# Autodesk Inventor assembly: Assy_wrist
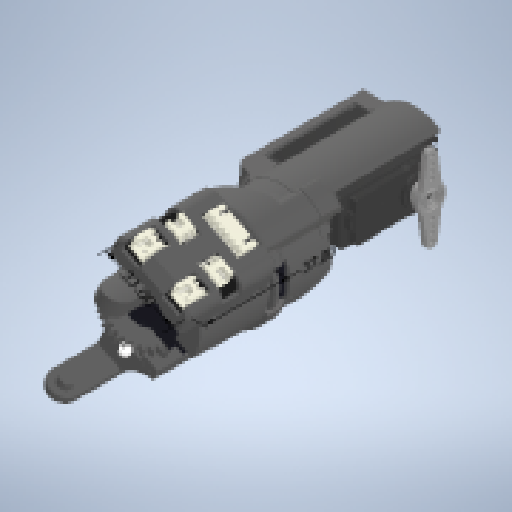
[picture p0: Inventor's stored thumbnail of the model, 512x512]
Saved by Autodesk Inventor 2024.1 (Build 281209000, 209)
## iProperties
Created: 2025-03-02
Part Number: Assy_wrist
Document SubType Name: Assembly
Designer: hibik
Author: hibik
## Documents named in this file (16)
- C:\Users\hibik\Documents\Robomech\RESCUE\ORCA\hard\arm\Assy_wrist.iam
- C:\Users\hibik\Documents\Robomech\RESCUE\ORCA\hard\arm\wrist_wrist.ipt
- C:\Users\hibik\Documents\Robomech\RESCUE\ORCA\hard\std_parts\Miusei_ms18.ipt
- C:\Users\hibik\Documents\Robomech\RESCUE\ORCA\hard\arm\hand_gear_wrist.ipt
- C:\Users\hibik\Documents\Robomech\RESCUE\ORCA\hard\std_parts\Miusei_hone_short.ipt
- C:\Users\hibik\Documents\Robomech\RESCUE\ORCA\hard\arm\wrist_hand_connector.ipt
- C:\Users\hibik\Documents\Robomech\RESCUE\ORCA\hard\arm\wrist_geard_hone.ipt
- C:\Users\hibik\Documents\Robomech\RESCUE\ORCA\hard\std_parts\bearing_6_10_3_MIR.ipt
- C:\Users\hibik\Documents\Robomech\RESCUE\ORCA\hard\arm\wrist_gear_spacer.ipt
- C:\Users\hibik\Documents\Robomech\RESCUE\ORCA\hard\arm\wrist_cover.ipt
- C:\Users\hibik\Documents\Robomech\RESCUE\ORCA\hard\std_parts\FS5103B.ipt
- C:\Users\hibik\Documents\Robomech\RESCUE\ORCA\hard\std_parts\feetech_servohone.ipt
- C:\Users\hibik\Documents\Robomech\RESCUE\ORCA\hard\arm\wrist_base.ipt
- C:\Users\hibik\Documents\Robomech\RESCUE\ORCA\hard\std_parts\bearing_6_10_3.ipt
- C:\Users\hibik\Documents\Robomech\RESCUE\ORCA\hard\board\CORE_model\md.iam
- C:\Users\hibik\Documents\Robomech\RESCUE\ORCA\hard\arm\wrist_board_cover.ipt
## Components (18 placed, 15 different names)
1. Miusei_ms18:1 — 挿入:1, メイト:7, メイト:8, メイト:9
2. hand_gear_wrist:1 — 挿入:2, 挿入:17
3. Miusei_hone_short:1 — 挿入:1, 挿入:2
4. wrist_hand_connector:1 — 挿入:15, 挿入:16
5. wrist_geard_hone:1 — 挿入:5, 挿入:11
6. bearing_6_10_3_MIR:1 — 挿入:5, 挿入:8
7. bearing_6_10_3_MIR:2 — 挿入:7
8. wrist_gear_spacer:1 — 挿入:7, 挿入:8
9. wrist_base:1 — 挿入:9, メイト:1, メイト:2, メイト:3, メイト:4, メイト:5, メイト:6, 挿入:12, 挿入:13
10. bearing_6_10_3:1 — 挿入:9
11. feetech_servohone:1 — 挿入:10
12. FS5103B:1 — 挿入:10, メイト:1, メイト:2, メイト:3
13. wrist_cover:1 — 挿入:12, 挿入:13, 挿入:14
14. wrist_wrist:1 — 挿入:14, 挿入:15, 挿入:16, メイト:7, メイト:8, メイト:9, 挿入:18, 角度:1, フラッシュ:1, フラッシュ:2, メイト:10
15. Miusei_ms18:2 — メイト:4, メイト:5, メイト:6, 挿入:11
16. bearing_6_10_3:2 — 挿入:17
17. md:1 [sub-assembly] — 挿入:18, 角度:1
18. wrist_board_cover:1 — フラッシュ:1, フラッシュ:2, メイト:10
## Relationships (28: Insert 15, Mate 10, Flush 2, Angle 1)
- 挿入:1 [Insert] (2 mm): Miusei_ms18:1 ↔ Miusei_hone_short:1
- 挿入:2 [Insert]: hand_gear_wrist:1 ↔ Miusei_hone_short:1
- 挿入:5 [Insert]: wrist_geard_hone:1 ↔ bearing_6_10_3_MIR:1
- 挿入:7 [Insert]: bearing_6_10_3_MIR:2 ↔ wrist_gear_spacer:1
- 挿入:8 [Insert]: bearing_6_10_3_MIR:1 ↔ wrist_gear_spacer:1
- 挿入:9 [Insert]: wrist_base:1 ↔ bearing_6_10_3:1
- 挿入:10 [Insert]: feetech_servohone:1 ↔ FS5103B:1
- メイト:1 [Mate]: wrist_base:1 ↔ FS5103B:1
- メイト:2 [Mate]: wrist_base:1 ↔ FS5103B:1
- メイト:3 [Mate]: wrist_base:1 ↔ FS5103B:1
- メイト:4 [Mate]: wrist_base:1 ↔ Miusei_ms18:2
- メイト:5 [Mate]: wrist_base:1 ↔ Miusei_ms18:2
- メイト:6 [Mate]: wrist_base:1 ↔ Miusei_ms18:2
- 挿入:11 [Insert]: wrist_geard_hone:1 ↔ Miusei_ms18:2
- 挿入:12 [Insert]: wrist_base:1 ↔ wrist_cover:1
- 挿入:13 [Insert]: wrist_base:1 ↔ wrist_cover:1
- 挿入:14 [Insert] (0.5 mm): wrist_cover:1 ↔ wrist_wrist:1
- 挿入:15 [Insert]: wrist_hand_connector:1 ↔ wrist_wrist:1
- 挿入:16 [Insert]: wrist_hand_connector:1 ↔ wrist_wrist:1
- メイト:7 [Mate]: Miusei_ms18:1 ↔ wrist_wrist:1
- メイト:8 [Mate]: Miusei_ms18:1 ↔ wrist_wrist:1
- メイト:9 [Mate]: Miusei_ms18:1 ↔ wrist_wrist:1
- 挿入:17 [Insert]: hand_gear_wrist:1 ↔ bearing_6_10_3:2
- 挿入:18 [Insert]: wrist_wrist:1 ↔ md:1
- 角度:1 [Angle] (0 deg): wrist_wrist:1 ↔ md:1
- フラッシュ:1 [Flush]: wrist_wrist:1 ↔ wrist_board_cover:1
- フラッシュ:2 [Flush]: wrist_wrist:1 ↔ wrist_board_cover:1
- メイト:10 [Mate] (8 mm): wrist_wrist:1 ↔ wrist_board_cover:1
